# Autodesk Inventor assembly: BGHK6800VV-30_MIR_CPY_MIR
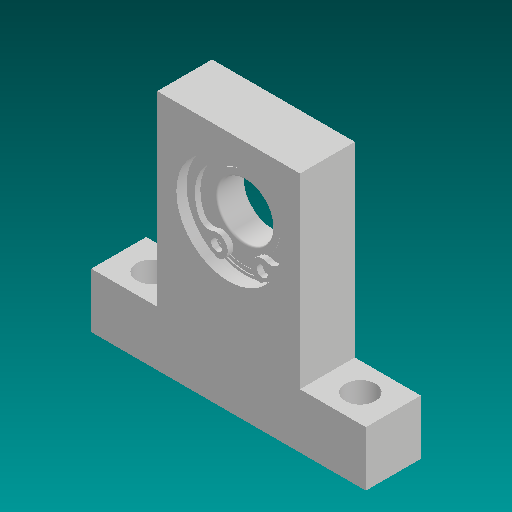
[picture p0: Inventor's stored thumbnail of the model, 512x512]
Saved by Autodesk Inventor 2020 (Build 240168000, 168)
## iProperties
Category: PARTsolutions
Company: MISUMI
Created: 2022-11-02
Part Number: BGHK6800VV-30_MIR_CPY_MIR
Catalog Web Link: www.cadenas.de
Description: BGHKB, BGHK, BGHKA, BGHKSA, BGHKS-Bearings with Housings T-Shaped h Selectable
Vendor: MISUMI
Document SubType Name: Assembly
Designer: kanazawakotaro
Manufacturer: MISUMI
Mass: 11.7791 g
Surface Area: 63.3194 cm^2
Volume: 11.7791 cm^3
Density: 1 g/cm^3
Title: BGHK6800VV-30
Author: Cadenas PARTsolutions
Comments: Bearings with Housings T-Shaped h Selectable
PSOL_IDENT_0: {$CADENAS_DATA/23d-libs/misumi/metric/12_bearing_holders/bghkb_asmtab.prj},241 {VTYP=3D},{STYP=ASSTA
PSOL_IDENT_1: B},{NB=BGHK6800VV-30},{LINA=BGHK6800VV-30},{NN=BGHKB, BGHK, BGHKA, BGHKSA, BGHKS},{DATE=30.06.2021 1
PSOL_IDENT_2: 2:58:11},{GEOMDATE=09.07.2015 08:06:15},{VERSION=},{LINEID=300},{WBVAR=MATB,MATH,STH,SEAL,HH,ALT1,AL
PSOL_IDENT_3: T2},{WBNUMERIC=HH}  {NB=BGHK6800VV-30},{LINA=BGHK6800VV-30},{KT=DUMMY},{PN=BGHK6800VV-30},{TYPE=BGHK
PSOL_IDENT_4: },{MATB=S},{MATBALG='S','Steel','SS','Stainless Steel'},{MATH=S45C},{MATHALG='S45C','1045 Carbon Ste
PSOL_IDENT_5: el','2017AA','2017 Aluminum Alloy'},{STH=ENP},{STHALG='BO','Black Oxide','ENP','Electroless Nickel P
PSOL_IDENT_6: lating'},{ARR=304 Stainless Steel},{ARR3D=-S},{BN=6800},{SEAL=VV},{SEALALG='ZZ','Double Shielded','V
PSOL_IDENT_7: V','Non-Contact Sealed Rubber Seal','DD','Contact Sealed Rubber Seal'},{HH=30},{HHALG=[20,25,30]},{D
PSOL_IDENT_8: D=10},{D=19},{DD2=20},{MM=1.15},{DDHH=16},{B=5},{LL1=2},{H=44},{H2=14},{L=50},{L1=38.0},{L2=26},{T=1
PSOL_IDENT_9: 0},{S=10},{DD1=5.5},{ALT1=},{ALT2=},{PPATH=bghkb/bghkb_asmtpl.prj}
NB: BGHK6800VV-30
NN: BGHKB, BGHK, BGHKA, BGHKSA, BGHKS
NT: Bearings with Housings T-Shaped h Selectable
NBSYN: $PN.
LINA: BGHK6800VV-30
CATALOG: Misumi
PN: BGHK6800VV-30
MATB: Steel
MATH: 1045 Carbon Steel
STH: Electroless Nickel Plating
ARR: 304 Stainless Steel
BN: 6800
SEAL: Non-Contact Sealed Rubber Seal
HH: 30
DD: 10
D: 19
DDHH: 16
B: 5
LL1: 2
H: 44
L: 50
L1: 38
L2: 26
T: 10
S: 10
DD1: 5.5
ALT1: Bearings, Retaining Rings Assembled
ALT2: w/o KCC (C2 Chamfer)
SUPPLIER: MISUMI
ARTICLENO: BGHK6800VV-30
BOMINFO: BGHK6800VV-30
CREATOR: CADENAS GmbH
## Documents named in this file (4)
- C:\Users\金澤航太郎\Documents\Inventor\kamuy2\Parts\BGHK6800VV-30_Autodesk_Inventor_2020_20221102\AIS2020\BGHK6800VV-30_MIR_CPY_MIR.iam
- C:\Users\金澤航太郎\Documents\Inventor\kamuy2\Parts\BGHK6800VV-30_Autodesk_Inventor_2020_20221102\AIS2020\BGHK6800VV-30_h_MIR_CPY_MIR.ipt
- C:\Users\金澤航太郎\Documents\Inventor\kamuy2\Parts\BGHK6800VV-30_Autodesk_Inventor_2020_20221102\AIS2020\bearing_6800_MIR_CPY_MIR.ipt
- C:\Users\金澤航太郎\Documents\Inventor\kamuy2\Parts\BGHK6800VV-30_Autodesk_Inventor_2020_20221102\AIS2020\RRING-C-INT-S-19_MIR_CPY_MIR.ipt
## Components (3 placed, 3 different names)
1. BGHK6800VV-30_h_MIR_CPY_MIR:1 — to_bearing_Z@1 <-> to_housing_Z@2, to_bearing_XY@1 <-> to_housing_XY@2, to_rring_Z@1 <-> rr_Z@3, to_rring_XY@1 <-> rr_XY@3, to_bearing_YZ@1 <-> to_housing_YZ@2, to_rring_YZ@1 <-> rr_YZ@3
2. bearing_6800_MIR_CPY_MIR:1 — to_bearing_Z@1 <-> to_housing_Z@2, to_bearing_XY@1 <-> to_housing_XY@2, to_bearing_YZ@1 <-> to_housing_YZ@2
3. RRING-C-INT-S-19_MIR_CPY_MIR:1 — to_rring_Z@1 <-> rr_Z@3, to_rring_XY@1 <-> rr_XY@3, to_rring_YZ@1 <-> rr_YZ@3
## Relationships (6: Mate 4, Angle 2)
- to_bearing_Z@1 <-> to_housing_Z@2 [Mate]: BGHK6800VV-30_h_MIR_CPY_MIR:1 ↔ bearing_6800_MIR_CPY_MIR:1
- to_bearing_XY@1 <-> to_housing_XY@2 [Mate]: BGHK6800VV-30_h_MIR_CPY_MIR:1 ↔ bearing_6800_MIR_CPY_MIR:1
- to_rring_Z@1 <-> rr_Z@3 [Mate]: BGHK6800VV-30_h_MIR_CPY_MIR:1 ↔ RRING-C-INT-S-19_MIR_CPY_MIR:1
- to_rring_XY@1 <-> rr_XY@3 [Mate]: BGHK6800VV-30_h_MIR_CPY_MIR:1 ↔ RRING-C-INT-S-19_MIR_CPY_MIR:1
- to_bearing_YZ@1 <-> to_housing_YZ@2 [Angle] (0 deg): BGHK6800VV-30_h_MIR_CPY_MIR:1 ↔ bearing_6800_MIR_CPY_MIR:1
- to_rring_YZ@1 <-> rr_YZ@3 [Angle] (0 deg): BGHK6800VV-30_h_MIR_CPY_MIR:1 ↔ RRING-C-INT-S-19_MIR_CPY_MIR:1
